# Autodesk Inventor assembly: total
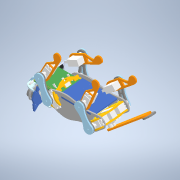
[picture p0: Inventor's stored thumbnail of the model, 180x180]
Saved by Autodesk Inventor 2020.3 (Build 243373000, 373)
## iProperties
Created: 2020-07-22
Part Number: total
Document SubType Name: Assembly
Designer: aditk
Author: aditk
## Documents named in this file (11)
- C:\Users\aditk\Desktop\PETcat\total.iam
- C:\Users\aditk\Desktop\PETcat\head _1_.iam
- C:\Users\aditk\Desktop\PETcat\leg1 _1_.iam
- C:\Users\aditk\Desktop\PETcat\body _1_.iam
- C:\Users\aditk\Desktop\PETcat\leg2 _1_.iam
- C:\Users\aditk\Desktop\PETcat\Part 14.ipt
- C:\Users\aditk\Desktop\PETcat\Part 15.ipt
- C:\Users\aditk\Desktop\PETcat\withsensors\20x40mm-rectangular-speaker-1.snapshot.1\20x40mm Rectangular Speaker\20x40mm Rectangular Speaker.ipt
- C:\Users\aditk\Desktop\PETcat\withsensors\16-channel-pwm-servo-controller-1.snapshot.2\Arduino 16 Channel PWM Module\12Channel PWM.ipt
- C:\Users\aditk\Desktop\PETcat\withsensors\mpu-9250-9dof-imu-1.snapshot.4\MPU-9250.ipt
- C:\Users\aditk\Desktop\PETcat\withsensors\raspberry-pi-4-b-work-in-progress-1.snapshot.6\Raspberry Pi 4 B.ipt
## Components (12 placed, 10 different names)
1. head _1_ [sub-assembly] — Insert:13, Mate:1
2. leg1 _1_ [sub-assembly] — Insert:11
3. body _1_ [sub-assembly] — Insert:2, Insert:4, Insert:9, Insert:11, Insert:12, Insert:13, Mate:2, Mate:3, Mate:5, Mate:7
4. leg2 _1_ [sub-assembly] — Insert:2
5. Part 14 — Insert:4, Insert:7
6. Part 15 — Insert:7
7. leg2 _1_:2 [sub-assembly] — Insert:9
8. leg1 _1_:2 [sub-assembly] — Insert:12
9. 20x40mm Rectangular Speaker:1 — Mate:1
10. 12Channel PWM:1 — Mate:4, Mate:5
11. MPU-9250:1 — Mate:6, Mate:7
12. Raspberry Pi 4 B:1 — Mate:2, Mate:3, Mate:4, Mate:6
## Relationships (14: Insert 7, Mate 7)
- Insert:2: body _1_ ↔ leg2 _1_
- Insert:4: body _1_ ↔ Part 14
- Insert:7: Part 14 ↔ Part 15
- Insert:9: body _1_ ↔ leg2 _1_:2
- Insert:11: leg1 _1_ ↔ body _1_
- Insert:12: body _1_ ↔ leg1 _1_:2
- Insert:13: head _1_ ↔ body _1_
- Mate:1: head _1_ ↔ 20x40mm Rectangular Speaker:1
- Mate:2: body _1_ ↔ Raspberry Pi 4 B:1
- Mate:3: body _1_ ↔ Raspberry Pi 4 B:1
- Mate:4 (10 mm): 12Channel PWM:1 ↔ Raspberry Pi 4 B:1
- Mate:5: body _1_ ↔ 12Channel PWM:1
- Mate:6 (10 mm): MPU-9250:1 ↔ Raspberry Pi 4 B:1
- Mate:7: body _1_ ↔ MPU-9250:1
